# Autodesk Inventor assembly: Force_plate
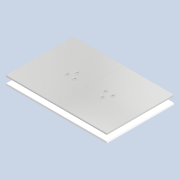
[picture p0: Inventor's stored thumbnail of the model, 180x180]
Saved by Autodesk Inventor 2022 (Build 260153000, 153)
## iProperties
Created: 2023-06-20
Part Number: Force_plate
Document SubType Name: Assembly
Designer: 81805
Author: 81805
## Documents named in this file (5)
- D:\GitHub\inventor\ForcePlate\Force_plate.iam
- D:\GitHub\inventor\ForcePlate\FFS080YS102U6.ipt
- D:\GitHub\inventor\ForcePlate\SFBJ6-8.ipt
- D:\GitHub\inventor\ForcePlate\Board.ipt
- D:\GitHub\inventor\ForcePlate\Bottom_board.ipt
## Components (11 placed, 4 different names)
1. FFS080YS102U6:1 — メイト:1, メイト:2, メイト:5
2. FFS080YS102U6:2 — メイト:3, メイト:4, メイト:6
3. SFBJ6-8:1 — 挿入:1
4. SFBJ6-8:2 — 挿入:2
5. SFBJ6-8:3 — 挿入:3
6. Board:1 — メイト:1, メイト:2, 挿入:1, 挿入:2, 挿入:3, フラッシュ:2, フラッシュ:3
7. Board:2 — メイト:3, メイト:4, 挿入:4, 挿入:5, 挿入:6, フラッシュ:1, フラッシュ:4
8. SFBJ6-8:4 — 挿入:6
9. SFBJ6-8:5 — 挿入:4
10. SFBJ6-8:6 — 挿入:5
11. Bottom_board:1 — メイト:5, メイト:6, フラッシュ:1, フラッシュ:2, フラッシュ:3, フラッシュ:4
## Relationships (16: Mate 6, Insert 6, Flush 4)
- メイト:1 [Mate]: FFS080YS102U6:1 ↔ Board:1
- メイト:2 [Mate]: FFS080YS102U6:1 ↔ Board:1
- メイト:3 [Mate]: FFS080YS102U6:2 ↔ Board:2
- メイト:4 [Mate]: FFS080YS102U6:2 ↔ Board:2
- 挿入:1 [Insert]: SFBJ6-8:1 ↔ Board:1
- 挿入:2 [Insert]: SFBJ6-8:2 ↔ Board:1
- 挿入:3 [Insert]: SFBJ6-8:3 ↔ Board:1
- 挿入:4 [Insert]: Board:2 ↔ SFBJ6-8:5
- 挿入:5 [Insert]: Board:2 ↔ SFBJ6-8:6
- 挿入:6 [Insert]: Board:2 ↔ SFBJ6-8:4
- メイト:5 [Mate]: FFS080YS102U6:1 ↔ Bottom_board:1
- メイト:6 [Mate]: FFS080YS102U6:2 ↔ Bottom_board:1
- フラッシュ:1 [Flush]: Board:2 ↔ Bottom_board:1
- フラッシュ:2 [Flush]: Board:1 ↔ Bottom_board:1
- フラッシュ:3 [Flush] (-0.25 mm): Board:1 ↔ Bottom_board:1
- フラッシュ:4 [Flush] (-0.25 mm): Board:2 ↔ Bottom_board:1
